# Autodesk Inventor assembly: Rr.wing_cradle
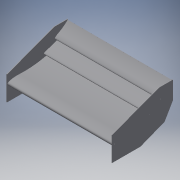
[picture p0: Inventor's stored thumbnail of the model, 180x180]
Saved by Autodesk Inventor 2018.2 (Build 222227000, 227)
## iProperties
Created: 2018-03-07
Part Number: Rr.wing_cradle
Material: 一般
Document SubType Name: Assembly
Designer: ku_sk
Author: ku_sk
## Documents named in this file (5)
- C:\Users\ku_sk\Documents\Inventor\Aero\KS-15\Rr.wing\cradle\base_model\Rr.wing_cradle\Rr.wing_cradle.iam
- C:\Users\ku_sk\Documents\Inventor\Aero\KS-15\Rr.wing\cradle\base_model\Rr.wing_cradle\parts\main frap.ipt
- C:\Users\ku_sk\Documents\Inventor\Aero\KS-15\Rr.wing\cradle\base_model\Rr.wing_cradle\parts\subflap.ipt
- C:\Users\ku_sk\Documents\Inventor\Aero\KS-15\Rr.wing\cradle\base_model\Rr.wing_cradle\parts\endplate.ipt
- C:\Users\ku_sk\Documents\Inventor\Aero\KS-15\Rr.wing\cradle\base_model\Rr.wing_cradle\parts\subflap(gurnee).ipt
## Components (5 placed, 4 different names)
1. main frap:1 — メイト:1, フラッシュ:1, メイト:2, メイト:3, メイト:4, メイト:5, 角度:1, 角度:2
2. subflap:1 — メイト:6, メイト:7, 角度:2, 角度:5
3. subflap(gurnee):1 — メイト:8, メイト:9, 角度:5
4. endplate:1 — メイト:3, メイト:4, フラッシュ:2, メイト:7, メイト:8
5. endplate:2 — メイト:2, メイト:5, フラッシュ:2, メイト:6, 角度:4, メイト:9
## Relationships (15: Mate 9, Angle 4, Flush 2)
- メイト:1 [Mate]: main frap:1
- フラッシュ:1 [Flush]: main frap:1
- メイト:2 [Mate]: main frap:1 ↔ endplate:2
- メイト:3 [Mate]: main frap:1 ↔ endplate:1
- メイト:4 [Mate]: main frap:1 ↔ endplate:1
- メイト:5 [Mate]: main frap:1 ↔ endplate:2
- フラッシュ:2 [Flush]: endplate:1 ↔ endplate:2
- メイト:6 [Mate]: subflap:1 ↔ endplate:2
- メイト:7 [Mate]: subflap:1 ↔ endplate:1
- 角度:1 [Angle] (15 deg): main frap:1
- 角度:2 [Angle] (-15 deg): main frap:1 ↔ subflap:1
- 角度:4 [Angle] (0 deg): endplate:2
- メイト:8 [Mate]: subflap(gurnee):1 ↔ endplate:1
- メイト:9 [Mate]: subflap(gurnee):1 ↔ endplate:2
- 角度:5 [Angle] (-15 deg): subflap:1 ↔ subflap(gurnee):1
